# Autodesk Inventor assembly: 바텀조립
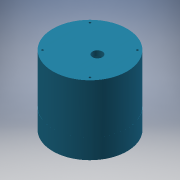
[picture p0: Inventor's stored thumbnail of the model, 180x180]
Saved by Autodesk Inventor 2019 (Build 230136000, 136)
## iProperties
Created: 2018-04-03
Part Number: 바텀조립
Material: 일반
Document SubType Name: Assembly
Designer: CK
Author: CK
## Documents named in this file (3)
- C:\Users\GMIMG\Documents\카카오톡 받은 파일\어셈파일\바텀조립.iam
- C:\Users\GMIMG\Documents\카카오톡 받은 파일\어셈파일\바텀(상).ipt
- C:\Users\GMIMG\Documents\카카오톡 받은 파일\어셈파일\바텀(하).ipt
## Components (2 placed, 2 different names)
1. 바텀(상):1 — 삽입:1
2. 바텀(하):1 — 삽입:1, 메이트:1
## Relationships (2: Insert 1, Mate 1)
- 삽입:1 [Insert]: 바텀(상):1 ↔ 바텀(하):1
- 메이트:1 [Mate]: 바텀(하):1
